# Autodesk Inventor assembly: Arm
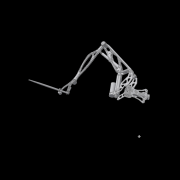
[picture p0: Inventor's stored thumbnail of the model, 180x180]
Saved by Autodesk Inventor 2020 (Build 240168000, 168)
## iProperties
Created: 2020-03-24
Part Number: Arm
Document SubType Name: Assembly
Designer: valer
Mass: 4853.13 g
Surface Area: 3141.52 cm^2
Volume: 1403.99 cm^3
Density: 3.45667 g/cm^3
Author: valer
## Documents named in this file (23)
- C:\Users\valer\Desktop\drummingrobot\src\parts\Arm.iam
- C:\Users\valer\Desktop\drummingrobot\src\parts\UpperArm.ipt
- C:\Users\valer\Desktop\drummingrobot\src\parts\UpperArmBracket.ipt
- C:\Users\valer\Desktop\drummingrobot\src\parts\Forearm.ipt
- C:\Users\valer\Desktop\drummingrobot\src\parts\external\Drumstick.ipt
- C:\Users\valer\Desktop\drummingrobot\src\parts\external\ForearmShaftCollar.ipt
- C:\Users\valer\Desktop\drummingrobot\src\parts\external\ArmSolenoid.ipt
- C:\Users\valer\Desktop\drummingrobot\src\parts\external\UpperArmActuatorBody.ipt
- C:\Users\valer\Desktop\drummingrobot\src\parts\external\UpperArmActuatorShaft.ipt
- C:\Users\valer\Desktop\drummingrobot\src\parts\external\ForearmActuatorBody.ipt
- C:\Users\valer\Desktop\drummingrobot\src\parts\external\ForearmActuatorShaft.ipt
- C:\Users\valer\Desktop\drummingrobot\src\parts\ForearmActuatorConnector.ipt
- C:\Users\valer\Desktop\drummingrobot\src\parts\SolenoidBracket.ipt
- C:\Users\valer\Desktop\drummingrobot\src\parts\external\ShoulderServo.ipt
- C:\Users\valer\Desktop\drummingrobot\src\parts\UpperArmShaftLock.ipt
- C:\Users\valer\Desktop\drummingrobot\src\parts\UpperArmBracketBase.ipt
- C:\Users\valer\Desktop\drummingrobot\src\parts\external\ShoulderMiterGear.ipt
- C:\Users\valer\Desktop\drummingrobot\src\parts\external\ShoulderServoShaft.ipt
- C:\Users\valer\Desktop\drummingrobot\src\parts\external\ServoShaft.ipt
- C:\Users\valer\Desktop\drummingrobot\src\parts\external\ShoulderMotorMount.ipt
- C:\Users\valer\Desktop\drummingrobot\src\parts\external\PatternSpacer.ipt
- C:\Users\valer\Desktop\drummingrobot\src\parts\ShoulderBracket2.ipt
- C:\Users\valer\Desktop\drummingrobot\src\parts\Potentiometer.iam
## Components (31 placed, 21 different names)
1. Drumstick:1 — Mate:79, Flush:3, Mate:292
2. ShaftCollar1/2:1 — Mate:79, Flush:3, Mate:236, Flush:18
3. ArmSolenoid:1 — Mate:290, Mate:291, Mate:292
4. UpperArmActuatorBody:1 — Mate:266, Mate:287
5. Forearm:1 — Flush:17, Mate:227, Mate:236, Flush:18, Mate:239, Mate:244, Mate:288, Mate:289
6. UpperArmActuatorShaft:2 — Mate:238, Flush:20, Mate:266
7. ForearmActuatorBody:1 — Mate:231, Mate:232, Mate:234, Flush:19
8. ForearmActuatorShaft:3 — Flush:17, Mate:231, Mate:232, Mate:241, Mate:243, Angle:10, Mate:246
9. UpperArm:3 — Mate:227, Mate:234, Mate:238, Flush:19, Flush:20, Mate:285, Mate:286, Mate:295, Mate:332, Mate:333, Mate:334, Mate:335
10. ForearmActuatorConnector:1 — Mate:239, Mate:241, Mate:245, Angle:10, Mate:246
11. ForearmActuatorConnector:2 — Mate:243, Mate:244, Mate:245
12. UpperArmBracket:5 — Mate:280, Mate:281, Mate:282, Mate:283, Mate:284
13. UpperArmBracket:6 — Mate:273, Mate:274, Mate:275, Mate:276, Mate:277, Mate:278, Mate:287
14. SolenoidBracket:1 — Mate:288, Mate:289, Mate:290, Mate:291
15. UpperArmShaftLock:1 — Mate:273, Mate:274, Mate:275, Mate:285, Mate:286
16. UpperArmBracketBase:1 — Mate:276, Mate:277, Mate:278, Mate:280, Mate:281, Mate:296, Angle:11, Mate:314, Mate:315
17. UpperArmShaftLock:2 — Mate:282, Mate:283, Mate:284, Mate:295
18. ShoulderServo:1 — Mate:301, Mate:302, Mate:340
19. ShoulderMiterGear:1 — Mate:303, Mate:317
20. ShoulderServoShaft:1 — Mate:301, Mate:302, Mate:303, Mate:316
21. ShoulderMiterGear:2 — Mate:296, Angle:11, Angle:12, Mate:318, Mate:339
22. ShoulderServoShaft:2 — Mate:314, Mate:315, Mate:319, Mate:320
23. ShoulderMotorMount:1 — Mate:316, Angle:12, Flush:24, Flush:26, Mate:326, Mate:327, Mate:340
24. ShoulderMotorMount:2 — Flush:25, Mate:319, Flush:26, Mate:321, Mate:322, Mate:323, Mate:324, Mate:325, Mate:328
25. PatternSpacer:1 — Mate:320, Mate:321, Mate:322
26. ShoulderBracket2:1 — Mate:323, Mate:324, Mate:325, Mate:331
27. ShoulderBracket2:2 — Mate:326, Mate:327, Mate:328, Mate:329, Mate:330
28. ShoulderMotorMount:3 — Mate:329, Mate:330, Mate:331, Mate:338
29. Potentiometer:1 [sub-assembly] — Mate:332, Mate:333
30. Potentiometer:2 [sub-assembly] — Mate:334, Mate:335
31. Potentiometer:3 [sub-assembly] — Mate:338, Mate:339
## Relationships (74: Mate 63, Flush 8, Angle 3)
- Mate:79: Drumstick:1 ↔ ShaftCollar1/2:1
- Flush:3 (304.8 mm): Drumstick:1 ↔ ShaftCollar1/2:1
- Flush:17: Forearm:1 ↔ ForearmActuatorShaft:3
- Mate:227: Forearm:1 ↔ UpperArm:3
- Mate:231: ForearmActuatorBody:1 ↔ ForearmActuatorShaft:3
- Mate:232: ForearmActuatorBody:1 ↔ ForearmActuatorShaft:3
- Mate:234: ForearmActuatorBody:1 ↔ UpperArm:3
- Mate:236: ShaftCollar1/2:1 ↔ Forearm:1
- Flush:18 (12.7 mm): ShaftCollar1/2:1 ↔ Forearm:1
- Mate:238: UpperArmActuatorShaft:2 ↔ UpperArm:3
- Flush:19: ForearmActuatorBody:1 ↔ UpperArm:3
- Flush:20: UpperArmActuatorShaft:2 ↔ UpperArm:3
- Mate:239: Forearm:1 ↔ ForearmActuatorConnector:1
- Mate:241: ForearmActuatorShaft:3 ↔ ForearmActuatorConnector:1
- Mate:243: ForearmActuatorShaft:3 ↔ ForearmActuatorConnector:2
- Mate:244: Forearm:1 ↔ ForearmActuatorConnector:2
- Mate:245: ForearmActuatorConnector:1 ↔ ForearmActuatorConnector:2
- Angle:10 (-180 deg): ForearmActuatorShaft:3 ↔ ForearmActuatorConnector:1
- Mate:246: ForearmActuatorShaft:3 ↔ ForearmActuatorConnector:1
- Mate:266: UpperArmActuatorBody:1 ↔ UpperArmActuatorShaft:2
- Mate:273: UpperArmBracket:6 ↔ UpperArmShaftLock:1
- Mate:274: UpperArmBracket:6 ↔ UpperArmShaftLock:1
- Mate:275: UpperArmBracket:6 ↔ UpperArmShaftLock:1
- Mate:276: UpperArmBracket:6 ↔ UpperArmBracketBase:1
- Mate:277: UpperArmBracket:6 ↔ UpperArmBracketBase:1
- Mate:278: UpperArmBracket:6 ↔ UpperArmBracketBase:1
- Mate:280: UpperArmBracket:5 ↔ UpperArmBracketBase:1
- Mate:281: UpperArmBracket:5 ↔ UpperArmBracketBase:1
- Mate:282: UpperArmBracket:5 ↔ UpperArmShaftLock:2
- Mate:283: UpperArmBracket:5 ↔ UpperArmShaftLock:2
- Mate:284: UpperArmBracket:5 ↔ UpperArmShaftLock:2
- Mate:285: UpperArm:3 ↔ UpperArmShaftLock:1
- Mate:286: UpperArm:3 ↔ UpperArmShaftLock:1
- Mate:287: UpperArmActuatorBody:1 ↔ UpperArmBracket:6
- Mate:288: Forearm:1 ↔ SolenoidBracket:1
- Mate:289: Forearm:1 ↔ SolenoidBracket:1
- Mate:290: ArmSolenoid:1 ↔ SolenoidBracket:1
- Mate:291: ArmSolenoid:1 ↔ SolenoidBracket:1
- Mate:292: Drumstick:1 ↔ ArmSolenoid:1
- Mate:295: UpperArm:3 ↔ UpperArmShaftLock:2
- Mate:296: UpperArmBracketBase:1 ↔ ShoulderMiterGear:2
- Angle:11 (0 deg): UpperArmBracketBase:1 ↔ ShoulderMiterGear:2
- Mate:301: ShoulderServo:1 ↔ ShoulderServoShaft:1
- Mate:302: ShoulderServo:1 ↔ ShoulderServoShaft:1
- Mate:303: ShoulderMiterGear:1 ↔ ShoulderServoShaft:1
- Mate:314: UpperArmBracketBase:1 ↔ ShoulderServoShaft:2
- Mate:315: UpperArmBracketBase:1 ↔ ShoulderServoShaft:2
- Mate:316: ShoulderServoShaft:1 ↔ ShoulderMotorMount:1
- Angle:12 (0 deg): ShoulderMiterGear:2 ↔ ShoulderMotorMount:1
- Flush:24: ShoulderMotorMount:1
- Mate:317 (1 mm): ShoulderMiterGear:1
- Mate:318 (1 mm): ShoulderMiterGear:2
- Flush:25: ShoulderMotorMount:2
- Mate:319: ShoulderServoShaft:2 ↔ ShoulderMotorMount:2
- Flush:26: ShoulderMotorMount:1 ↔ ShoulderMotorMount:2
- Mate:320: ShoulderServoShaft:2 ↔ PatternSpacer:1
- Mate:321: ShoulderMotorMount:2 ↔ PatternSpacer:1
- Mate:322: ShoulderMotorMount:2 ↔ PatternSpacer:1
- Mate:323: ShoulderMotorMount:2 ↔ ShoulderBracket2:1
- Mate:324: ShoulderMotorMount:2 ↔ ShoulderBracket2:1
- Mate:325: ShoulderMotorMount:2 ↔ ShoulderBracket2:1
- Mate:326: ShoulderMotorMount:1 ↔ ShoulderBracket2:2
- Mate:327: ShoulderMotorMount:1 ↔ ShoulderBracket2:2
- Mate:328: ShoulderMotorMount:2 ↔ ShoulderBracket2:2
- Mate:329: ShoulderBracket2:2 ↔ ShoulderMotorMount:3
- Mate:330: ShoulderBracket2:2 ↔ ShoulderMotorMount:3
- Mate:331: ShoulderBracket2:1 ↔ ShoulderMotorMount:3
- Mate:332: UpperArm:3 ↔ Potentiometer:1
- Mate:333: UpperArm:3 ↔ Potentiometer:1
- Mate:334: UpperArm:3 ↔ Potentiometer:2
- Mate:335: UpperArm:3 ↔ Potentiometer:2
- Mate:338: ShoulderMotorMount:3 ↔ Potentiometer:3
- Mate:339: ShoulderMiterGear:2 ↔ Potentiometer:3
- Mate:340 (2 mm): ShoulderServo:1 ↔ ShoulderMotorMount:1
